# Autodesk Inventor assembly: Box Arm
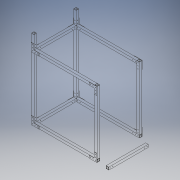
[picture p0: Inventor's stored thumbnail of the model, 180x180]
Saved by Autodesk Inventor 2018 (Build 220112000, 112)
## iProperties
Created: 2019-01-16
Part Number: Box Arm
Document SubType Name: Assembly
Designer: Gabriel
Author: Gabriel
## Documents named in this file (6)
- C:\Users\Gabriel\Documents\Drivebase Box Arm\Box Arm.iam
- C:\Users\Gabriel\Documents\Drivebase Box Arm\30in 1x1 Beam.ipt
- C:\Users\Gabriel\Documents\Drivebase Box Arm\25in 1x1 Beam.ipt
- C:\Users\Gabriel\Documents\Drivebase Box Arm\17in 1x1 Beam.ipt
- C:\Users\Gabriel\Documents\Drivebase Box Arm\23in 1x1 Beam.ipt
- C:\Users\Gabriel\Documents\Drivebase Box Arm\L gusset.ipt
## Components (23 placed, 5 different names)
1. 30in 1x1 Beam:1 — Mate:7, Mate:8, Mate:13, Mate:14, Mate:35, Mate:36, Mate:37, Mate:38
2. 30in 1x1 Beam:2 — Mate:5, Mate:6, Mate:11, Mate:12, Mate:33, Mate:34, Mate:39, Mate:40
3. 25in 1x1 Beam:1 — Mate:57, Mate:58, Mate:59, Mate:60
4. 25in 1x1 Beam:2 — Mate:61, Mate:62, Mate:63, Mate:64
5. 25in 1x1 Beam:3 — Mate:29, Mate:30, Mate:53, Mate:54
6. 25in 1x1 Beam:4 — Mate:31, Mate:32, Mate:55, Mate:56
7. 17in 1x1 Beam:1
8. 17in 1x1 Beam:2 — Mate:21, Mate:22, Mate:23, Mate:24
9. 17in 1x1 Beam:4 — Mate:41, Mate:42, Mate:45, Mate:46
10. 23in 1x1 Beam:1 — Mate:43, Mate:44, Mate:49, Mate:50
11. 23in 1x1 Beam:2 — Mate:47, Mate:48, Mate:51, Mate:52
12. L gusset:1 — Mate:53, Mate:54, Mate:63, Mate:64
13. L gusset:4 — Mate:49, Mate:50, Mate:61, Mate:62
14. L gusset:5 — Mate:51, Mate:52, Mate:57, Mate:58
15. L gusset:7 — Mate:11, Mate:12, Mate:23, Mate:24
16. L gusset:9 — Mate:13, Mate:14, Mate:21, Mate:22
17. L gusset:11 — Mate:7, Mate:8, Mate:31, Mate:32
18. L gusset:12 — Mate:5, Mate:6, Mate:29, Mate:30
19. L gusset:13 — Mate:33, Mate:34, Mate:43, Mate:44
20. L gusset:14 — Mate:35, Mate:36, Mate:47, Mate:48
21. L gusset:15 — Mate:39, Mate:40, Mate:42, Mate:45
22. L gusset:16 — Mate:37, Mate:38, Mate:41, Mate:46
23. L gusset:17 — Mate:55, Mate:56, Mate:59, Mate:60
## Relationships (48: Mate 48)
- Mate:5: 30in 1x1 Beam:2 ↔ L gusset:12
- Mate:6: 30in 1x1 Beam:2 ↔ L gusset:12
- Mate:7: 30in 1x1 Beam:1 ↔ L gusset:11
- Mate:8: 30in 1x1 Beam:1 ↔ L gusset:11
- Mate:11: 30in 1x1 Beam:2 ↔ L gusset:7
- Mate:12: 30in 1x1 Beam:2 ↔ L gusset:7
- Mate:13: 30in 1x1 Beam:1 ↔ L gusset:9
- Mate:14: 30in 1x1 Beam:1 ↔ L gusset:9
- Mate:21: 17in 1x1 Beam:2 ↔ L gusset:9
- Mate:22: 17in 1x1 Beam:2 ↔ L gusset:9
- Mate:23: 17in 1x1 Beam:2 ↔ L gusset:7
- Mate:24: 17in 1x1 Beam:2 ↔ L gusset:7
- Mate:29: 25in 1x1 Beam:3 ↔ L gusset:12
- Mate:30: 25in 1x1 Beam:3 ↔ L gusset:12
- Mate:31: 25in 1x1 Beam:4 ↔ L gusset:11
- Mate:32: 25in 1x1 Beam:4 ↔ L gusset:11
- Mate:33: 30in 1x1 Beam:2 ↔ L gusset:13
- Mate:34: 30in 1x1 Beam:2 ↔ L gusset:13
- Mate:35: 30in 1x1 Beam:1 ↔ L gusset:14
- Mate:36: 30in 1x1 Beam:1 ↔ L gusset:14
- Mate:37: 30in 1x1 Beam:1 ↔ L gusset:16
- Mate:38: 30in 1x1 Beam:1 ↔ L gusset:16
- Mate:39: 30in 1x1 Beam:2 ↔ L gusset:15
- Mate:40: 30in 1x1 Beam:2 ↔ L gusset:15
- Mate:41: 17in 1x1 Beam:4 ↔ L gusset:16
- Mate:42: 17in 1x1 Beam:4 ↔ L gusset:15
- Mate:43: 23in 1x1 Beam:1 ↔ L gusset:13
- Mate:44: 23in 1x1 Beam:1 ↔ L gusset:13
- Mate:45: 17in 1x1 Beam:4 ↔ L gusset:15
- Mate:46: 17in 1x1 Beam:4 ↔ L gusset:16
- Mate:47: 23in 1x1 Beam:2 ↔ L gusset:14
- Mate:48: 23in 1x1 Beam:2 ↔ L gusset:14
- Mate:49: 23in 1x1 Beam:1 ↔ L gusset:4
- Mate:50: 23in 1x1 Beam:1 ↔ L gusset:4
- Mate:51: 23in 1x1 Beam:2 ↔ L gusset:5
- Mate:52: 23in 1x1 Beam:2 ↔ L gusset:5
- Mate:53: 25in 1x1 Beam:3 ↔ L gusset:1
- Mate:54: 25in 1x1 Beam:3 ↔ L gusset:1
- Mate:55: 25in 1x1 Beam:4 ↔ L gusset:17
- Mate:56: 25in 1x1 Beam:4 ↔ L gusset:17
- Mate:57: 25in 1x1 Beam:1 ↔ L gusset:5
- Mate:58: 25in 1x1 Beam:1 ↔ L gusset:5
- Mate:59: 25in 1x1 Beam:1 ↔ L gusset:17
- Mate:60: 25in 1x1 Beam:1 ↔ L gusset:17
- Mate:61: 25in 1x1 Beam:2 ↔ L gusset:4
- Mate:62: 25in 1x1 Beam:2 ↔ L gusset:4
- Mate:63: 25in 1x1 Beam:2 ↔ L gusset:1
- Mate:64: 25in 1x1 Beam:2 ↔ L gusset:1
